# Autodesk Inventor assembly: BRAIN-assembly-complete-model-08-13-18
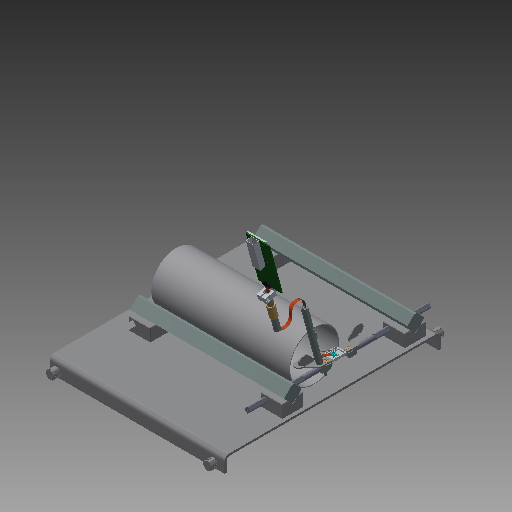
[picture p0: Inventor's stored thumbnail of the model, 512x512]
Saved by Autodesk Inventor 2019 (Build 230136000, 136)
## iProperties
Created: 2018-06-26
Part Number: BRAIN-assembly-complete-model-08-13-18
Description: Creo Elements/Direct Modeling STEP Export
Document SubType Name: Assembly
Designer: Brian
Sending System: PTC Creo Elements/Direct Modeling 19.0C  15-Aug-2015 (C) Parametric Technology GmbH
Preprocessor: PTC Creo Elements/Direct Modeling STEP processor for AP214 (Solid Model)
Title: BRAIN-assembly-complete-model-06-26-18.stp
## Documents named in this file (9)
- C:\Users\bgereke\Desktop\designs\Nord\BRAIN-assembly-complete-model-08-13-18.iam
- C:\Users\bgereke\Desktop\designs\Nord\Data-collection-assembly.iam
- C:\Users\bgereke\Desktop\designs\Nord\Head-Clamp-monolith-clamp-V2-RH.1.ipt
- C:\Users\bgereke\Desktop\designs\Nord\A-P-bar-01.ipt
- C:\Users\bgereke\Desktop\designs\Nord\A-P-bar-02.ipt
- C:\Users\bgereke\Desktop\designs\Nord\EarBar-02b.ipt
- C:\Users\bgereke\Desktop\designs\Nord\EarBar-01b.ipt
- C:\Users\bgereke\Desktop\designs\Nord\Mammock-assembly.iam
- C:\Users\bgereke\Desktop\designs\rat_cylinder.ipt
## Components (8 placed, 8 different names)
1. Data-collection-assembly_314 [sub-assembly] — Mate:2, Flush:1, Flush:2, Mate:3, Mate:4, Mate:5, Mate:6, Mate:7, Mate:8, Flush:9
2. Head-Clamp-monolith-clamp-V2-RH.1:1 — Mate:2, Mate:6, Mate:7
3. A-P-bar-01_39 — Flush:1, Flush:4, Flush:6, Mate:4, Mate:5, Mate:9, Mate:10, Flush:7
4. A-P-bar-02_36 — Flush:2, Flush:3, Flush:6, Mate:8, Flush:8, Mate:11, Mate:12
5. EarBar-02b_37 — Flush:3, Flush:8, Mate:11, Mate:12
6. EarBar-01b_41 — Flush:4, Mate:9, Mate:10, Flush:7
7. Mammock-assembly_311 [sub-assembly] — Mate:3, Flush:9
8. rat_cylinder:1
## Relationships (19: Mate 11, Flush 8)
- Mate:2: Data-collection-assembly_314 ↔ Head-Clamp-monolith-clamp-V2-RH.1:1
- Flush:1: Data-collection-assembly_314 ↔ A-P-bar-01_39
- Flush:2: Data-collection-assembly_314 ↔ A-P-bar-02_36
- Flush:3: A-P-bar-02_36 ↔ EarBar-02b_37
- Flush:4: A-P-bar-01_39 ↔ EarBar-01b_41
- Mate:3: Data-collection-assembly_314 ↔ Mammock-assembly_311
- Flush:6: A-P-bar-01_39 ↔ A-P-bar-02_36
- Mate:4: Data-collection-assembly_314 ↔ A-P-bar-01_39
- Mate:5: Data-collection-assembly_314 ↔ A-P-bar-01_39
- Mate:6: Data-collection-assembly_314 ↔ Head-Clamp-monolith-clamp-V2-RH.1:1
- Mate:7: Data-collection-assembly_314 ↔ Head-Clamp-monolith-clamp-V2-RH.1:1
- Mate:8: Data-collection-assembly_314 ↔ A-P-bar-02_36
- Mate:9: A-P-bar-01_39 ↔ EarBar-01b_41
- Mate:10: A-P-bar-01_39 ↔ EarBar-01b_41
- Flush:7: A-P-bar-01_39 ↔ EarBar-01b_41
- Flush:8: A-P-bar-02_36 ↔ EarBar-02b_37
- Mate:11: A-P-bar-02_36 ↔ EarBar-02b_37
- Mate:12: A-P-bar-02_36 ↔ EarBar-02b_37
- Flush:9 (52.7 mm): Data-collection-assembly_314 ↔ Mammock-assembly_311
